# Autodesk Inventor assembly: complete
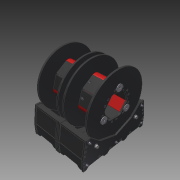
[picture p0: Inventor's stored thumbnail of the model, 180x180]
Saved by Autodesk Inventor 2014 (Build 180170000, 170)
## iProperties
Created: 2014-04-08
Part Number: complete
Document SubType Name: Assembly
Designer: buben
Author: buben
## Documents named in this file (3)
- C:\Users\buben\Documents\GitHub\bspool\inventor_files\assemblies\complete.iam
- C:\Users\buben\Documents\GitHub\bspool\inventor_files\assemblies\spool.iam
- C:\Users\buben\Documents\GitHub\bspool\inventor_files\assemblies\spool_stand.iam
## Components (3 placed, 2 different names)
1. spool:1 [sub-assembly] — Flush:1, Flush:2, Mate:4, Tangent:1, Tangent:2
2. spool:2 [sub-assembly] — Flush:1, Flush:2, Mate:5
3. spool_stand:1 [sub-assembly] — Mate:1, Mate:2, Mate:3, Mate:4, Tangent:1, Tangent:2, Mate:5
## Relationships (9: Mate 5, Flush 2, Tangent 2)
- Mate:1: spool_stand:1
- Mate:2: spool_stand:1
- Mate:3: spool_stand:1
- Flush:1: spool:1 ↔ spool:2
- Flush:2: spool:1 ↔ spool:2
- Mate:4 (1 mm): spool:1 ↔ spool_stand:1
- Tangent:1: spool:1 ↔ spool_stand:1
- Tangent:2: spool:1 ↔ spool_stand:1
- Mate:5 (1 mm): spool:2 ↔ spool_stand:1
